# Autodesk Inventor assembly: SARC315
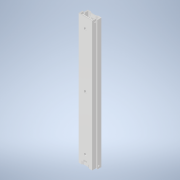
[picture p0: Inventor's stored thumbnail of the model, 180x180]
Saved by Autodesk Inventor 2022 (Build 260153000, 153)
## iProperties
Company: CADENAS
Created: 2022-02-05
Part Number: SARC315
Description: STEP AP203
Document SubType Name: Assembly
Designer: YusukeKunita
Sending System: PARTsolutions
Title: e:/temp/worker_26/temp/exporttempdir_412_452_QhePu/format_0/SARC315.stp
Author: License CC BY-ND 4.0
Revision Number: NONE
## Documents named in this file (4)
- C:\Users\YusukeKunita\Documents\GrabCAD\NHK2022\BasicParts\SlideRail\SARC315\SARC315.iam
- C:\Users\YusukeKunita\Documents\GrabCAD\NHK2022\BasicParts\SlideRail\SARC315\_SARC315_or.ipt
- C:\Users\YusukeKunita\Documents\GrabCAD\NHK2022\BasicParts\SlideRail\SARC315\_SARC315_re.ipt
- C:\Users\YusukeKunita\Documents\GrabCAD\NHK2022\BasicParts\SlideRail\SARC315\_SARC315_ir.ipt
## Components (5 placed, 5 different names)
1. NAUO1 — メイト:1, 正接:1, 正接:2, フラッシュ:1, フラッシュ:2
2. NAUO2 — メイト:1, 正接:1, 正接:2, メイト:2, 正接:3, 正接:4, 円柱状:1
3. NAUO3 — メイト:2, 正接:3, 正接:4, 円柱状:1, メイト:3, 正接:6, 正接:10, 円柱状:2, フラッシュ:2, フラッシュ:3
4. NAUO4 — メイト:4, 正接:7, 正接:9, メイト:3, 正接:6, 正接:10, 円柱状:2
5. NAUO5 — メイト:4, 正接:7, 正接:9, フラッシュ:1, フラッシュ:3
## Relationships (17: Tangent 8, Mate 4, Flush 3, CylindricalJoint 2)
- メイト:1 [Mate] (0.5 mm): NAUO1 ↔ NAUO2
- 正接:1 [Tangent]: NAUO1 ↔ NAUO2
- 正接:2 [Tangent]: NAUO1 ↔ NAUO2
- メイト:2 [Mate] (0.3 mm): NAUO2 ↔ NAUO3
- 正接:3 [Tangent]: NAUO2 ↔ NAUO3
- 正接:4 [Tangent]: NAUO2 ↔ NAUO3
- 円柱状:1 [CylindricalJoint]: NAUO2 ↔ NAUO3
- メイト:4 [Mate] (0.5 mm): NAUO4 ↔ NAUO5
- 正接:7 [Tangent]: NAUO4 ↔ NAUO5
- 正接:9 [Tangent]: NAUO4 ↔ NAUO5
- メイト:3 [Mate] (0.3 mm): NAUO3 ↔ NAUO4
- 正接:6 [Tangent]: NAUO3 ↔ NAUO4
- 正接:10 [Tangent]: NAUO3 ↔ NAUO4
- 円柱状:2 [CylindricalJoint]: NAUO3 ↔ NAUO4
- フラッシュ:1 [Flush]: NAUO1 ↔ NAUO5
- フラッシュ:2 [Flush]: NAUO1 ↔ NAUO3
- フラッシュ:3 [Flush]: NAUO3 ↔ NAUO5
